# Autodesk Inventor assembly: populated-keyboard_cherrymx
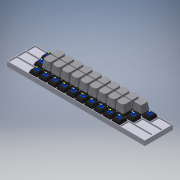
[picture p0: Inventor's stored thumbnail of the model, 180x180]
Saved by Autodesk Inventor 2016 (Build 200138000, 138)
## iProperties
Created: 2016-12-08
Part Number: populated-keyboard_cherrymx
Document SubType Name: Assembly
Designer: Cemra JC
Author: Cemra JC
## Documents named in this file (3)
- J:\The Files\The Software Files\Projects\stenotoppers\cherrymx\base-model\populated-keyboard_cherrymx.iam
- J:\The Files\The Software Files\Projects\stenotoppers\cherrymx\base-model\keyboard-mockup_cherrymx.iam
- J:\The Files\The Software Files\Projects\stenotoppers\cherrymx\base-model\standard-keycap_top-rows_base_cherrymx.ipt
## Components (20 placed, 2 different names)
1. keyboard-mockup_cherrymx:1 [sub-assembly] — Rigid:2, Rigid:3
2. standard-keycap_top-rows_base_cherrymx:4 — Rigid:3
3. standard-keycap_top-rows_base_cherrymx:5
4. standard-keycap_top-rows_base_cherrymx:6
5. standard-keycap_top-rows_base_cherrymx:7
6. standard-keycap_top-rows_base_cherrymx:8
7. standard-keycap_top-rows_base_cherrymx:9
8. standard-keycap_top-rows_base_cherrymx:10
9. standard-keycap_top-rows_base_cherrymx:11
10. standard-keycap_top-rows_base_cherrymx:12
11. standard-keycap_top-rows_base_cherrymx:13
12. standard-keycap_top-rows_base_cherrymx:2 — Rigid:2
13. standard-keycap_top-rows_base_cherrymx:14
14. standard-keycap_top-rows_base_cherrymx:15
15. standard-keycap_top-rows_base_cherrymx:16
16. standard-keycap_top-rows_base_cherrymx:17
17. standard-keycap_top-rows_base_cherrymx:18
18. standard-keycap_top-rows_base_cherrymx:19
19. standard-keycap_top-rows_base_cherrymx:20
20. standard-keycap_top-rows_base_cherrymx:21
## Component patterns: (10 elements, first: standard-keycap_top-rows_base_cherrymx:4), (9 elements, first: standard-keycap_top-rows_base_cherrymx:2)
## Relationships (2: WeldJoint 2)
- Rigid:2 [WeldJoint]: keyboard-mockup_cherrymx:1 ↔ standard-keycap_top-rows_base_cherrymx:2
- Rigid:3 [WeldJoint]: keyboard-mockup_cherrymx:1 ↔ standard-keycap_top-rows_base_cherrymx:4
